# Autodesk Inventor assembly: HousingAssemblyV2
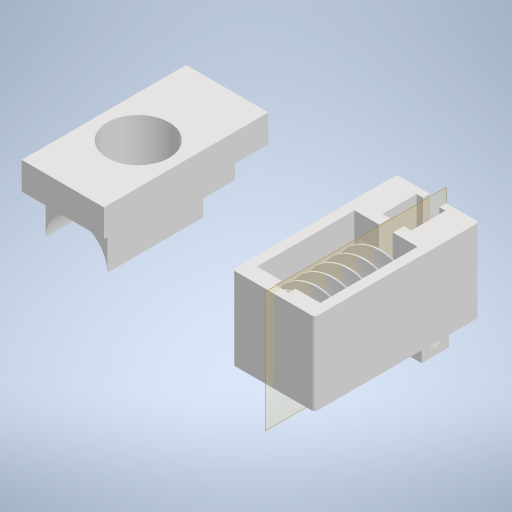
[picture p0: Inventor's stored thumbnail of the model, 512x512]
Saved by Autodesk Inventor 2023 (Build 270158000, 158)
## iProperties
Created: 2023-04-05
Part Number: HousingAssemblyV2
Document SubType Name: Assembly
Designer: czapa
Author: czapa
## Documents named in this file (4)
- C:\Users\czapa\OneDrive\Documents\GitHub\S.P.I.C.E\3D Models\Version1\HousingAssemblyV2.iam
- C:\Users\czapa\OneDrive\Documents\GitHub\S.P.I.C.E\3D Models\housing_V3.ipt
- C:\Users\czapa\OneDrive\Documents\GitHub\S.P.I.C.E\3D Models\housing_lid_V3.ipt
- C:\Users\czapa\OneDrive\Documents\GitHub\S.P.I.C.E\3D Models\spiralV2.ipt
## Components (3 placed, 3 different names)
1. housing_V3:1 — Mate:1
2. housing_lid_V3:1
3. spiralV2:1 — Mate:1
## Relationships (1: Mate 1)
- Mate:1: housing_V3:1 ↔ spiralV2:1
